# Autodesk Inventor assembly: 093
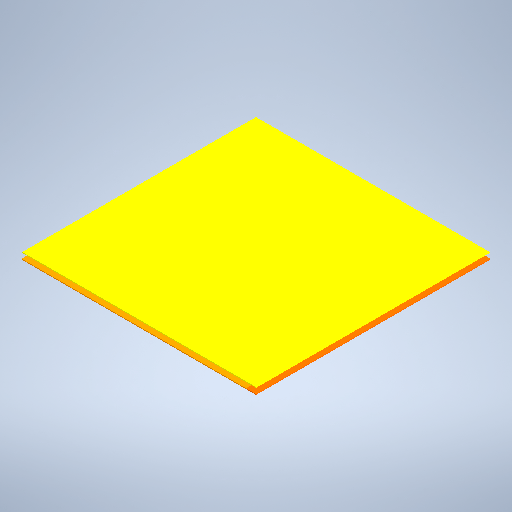
[picture p0: Inventor's stored thumbnail of the model, 512x512]
Saved by Autodesk Inventor 2026 (Build 300175000, 175)
## iProperties
Created: 2026-05-19
Part Number: 093
Document SubType Name: Assembly
Designer: user
Author: user
## Documents named in this file (4)
- C:\Users\user\Documents\Inventor\GBK-Gubkinskiy\093.iam
- C:\Users\user\Documents\Inventor\GBK-Gubkinskiy\0931.ipt
- C:\Users\user\Documents\Inventor\GBK-Gubkinskiy\0932.ipt
- C:\Users\user\Documents\Inventor\GBK-Gubkinskiy\0933.ipt
## Components (3 placed, 3 different names)
1. 0931:1 — Совмещение:1, Заподлицо:1, Заподлицо:2
2. 0932:1 — Жесткий:1, Совмещение:1, Заподлицо:1
3. 0933:1 — Жесткий:1, Заподлицо:2
## Relationships (4: Flush 2, WeldJoint 1, Mate 1)
- Жесткий:1 [WeldJoint]: 0932:1 ↔ 0933:1
- Совмещение:1 [Mate]: 0931:1 ↔ 0932:1
- Заподлицо:1 [Flush] (34 mm): 0931:1 ↔ 0932:1
- Заподлицо:2 [Flush] (34 mm): 0931:1 ↔ 0933:1
